# Autodesk Inventor assembly: robot2
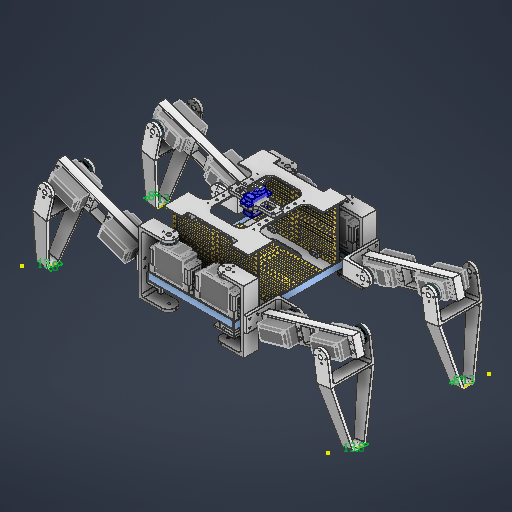
[picture p0: Inventor's stored thumbnail of the model, 512x512]
Saved by Autodesk Inventor 2026.1 (Build 301233000, 233)
## iProperties
Created: 2025-10-04
Part Number: robot2
Document SubType Name: Assembly
Designer: emanuel
Author: emanuel
## Documents named in this file (18)
- C:\Users\emanuel\UnFolder\SpiderRobo\3dmodel\robot2.iam
- C:\Users\emanuel\UnFolder\SpiderRobo\3dmodel\aluminium_profile_1.ipt
- C:\Users\emanuel\UnFolder\SpiderRobo\3dmodel\aluminium_profile_2.ipt
- C:\Users\emanuel\UnFolder\SpiderRobo\3dmodel\mg996r.ipt
- C:\Users\emanuel\UnFolder\SpiderRobo\3dmodel\support_2_servos.ipt
- C:\Users\emanuel\UnFolder\SpiderRobo\3dmodel\servo_disc.ipt
- C:\Users\emanuel\UnFolder\SpiderRobo\3dmodel\servo_support_4.ipt
- C:\Users\emanuel\UnFolder\SpiderRobo\3dmodel\small_bearing.ipt
- C:\Users\emanuel\UnFolder\SpiderRobo\3dmodel\underplate_support_1.ipt
- C:\Users\emanuel\UnFolder\SpiderRobo\3dmodel\bearing_support.ipt
- C:\Users\emanuel\UnFolder\SpiderRobo\3dmodel\C1.ipt
- C:\Users\emanuel\UnFolder\SpiderRobo\3dmodel\femur.ipt
- C:\Users\emanuel\UnFolder\SpiderRobo\3dmodel\L2.ipt
- C:\Users\emanuel\UnFolder\SpiderRobo\3dmodel\smart_calf.ipt
- C:\Users\emanuel\UnFolder\SpiderRobo\3dmodel\yellow_base.iam
- C:\Users\emanuel\UnFolder\SpiderRobo\3dmodel\base.ipt
- C:\Users\emanuel\UnFolder\SpiderRobo\3dmodel\sg90.ipt
- C:\Users\emanuel\UnFolder\SpiderRobo\3dmodel\microservo_support1.ipt
## Components (67 placed, 17 different names)
1. support_2_servos:1 — Mate:9, Flush:5, Mate:10, Mate:25, Flush:13, Flush:14, Mate:26, Flush:15, Flush:16, Mate:27, Flush:17, Flush:18, Mate:28, Flush:19, Flush:20
2. support_2_servos:2 — Mate:7, Flush:4, Mate:8, Mate:20, Mate:21, Flush:6, Mate:22, Flush:7, Flush:8, Mate:23, Flush:9, Flush:10, Mate:24, Flush:11, Flush:12
3. aluminium_profile_1:1 — Mate:3, Mate:4, Flush:2, Mate:5, Flush:3, Mate:7, Mate:43, Flush:22, Mate:46, Flush:25, Mate:128, Mate:134
4. aluminium_profile_1:2 — Mate:1, Mate:2, Flush:1, Mate:6, Mate:9, Mate:44, Flush:23, Mate:45, Flush:27, Mate:127, Mate:132, Mate:137
5. aluminium_profile_2:1 — Mate:5, Mate:6, Flush:3, Flush:4, Mate:8, Flush:26, Flush:28
6. aluminium_profile_2:2 — Mate:1, Mate:2, Flush:1, Mate:3, Mate:4, Flush:2, Flush:5, Mate:10, Flush:21, Flush:24
7. mg996r:1 — Mate:11, Mate:12, Mate:34, Mate:35, Mate:36
8. servo_disc:1 — Mate:11, Mate:12, Mate:49, Mate:51, Mate:52
9. mg996r:2 — Mate:40, Mate:41, Mate:42
10. servo_disc:2 — Mate:79, Mate:80
11. mg996r:3 — Mate:37, Mate:38, Mate:39
12. servo_disc:3 — Mate:69, Mate:70
13. servo_support_4:1 — Mate:28, Flush:19, Flush:20
14. servo_support_4:2 — Mate:26, Flush:15, Flush:16, Mate:34, Mate:35, Mate:36
15. servo_support_4:3 — Mate:27, Flush:17, Flush:18, Mate:31, Mate:32, Mate:33
16. servo_support_4:4 — Mate:25, Flush:13, Flush:14
17. servo_support_4:9 — Mate:20, Mate:21, Flush:6
18. servo_support_4:10 — Mate:23, Flush:9, Flush:10, Mate:37, Mate:38, Mate:39
19. servo_support_4:11 — Mate:22, Flush:7, Flush:8, Mate:40, Mate:41, Mate:42
20. servo_support_4:12 — Mate:24, Flush:11, Flush:12
21. mg996r:4 — Mate:31, Mate:32, Mate:33
22. servo_disc:4 — Mate:77, Mate:78
23. underplate_support_1:1 — Mate:43, Flush:21, Flush:22, Mate:50, Flush:29, Flush:30
24. underplate_support_1:2 — Mate:44, Flush:23, Flush:24
25. underplate_support_1:3 — Mate:46, Flush:25, Flush:26
26. underplate_support_1:4 — Mate:45, Flush:27, Flush:28
27. small_bearing:1 — Mate:49
28. bearing_support:1 — Mate:50, Flush:29, Flush:30
29. C1:1 — Mate:51, Mate:52, Mate:63, Mate:64, Mate:65, Mate:129
30. mg996r:5 — Mate:53, Mate:54, Mate:57, Mate:58, Mate:59
31. femur:1 — Mate:57, Mate:58, Mate:59, Mate:60, Mate:61, Mate:62
32. L2:1 — Mate:63, Mate:64, Mate:65, Mate:119, Mate:120
33. servo_disc:5 — Mate:53, Mate:54, Mate:125, Mate:126
34. mg996r:6 — Mate:60, Mate:61, Mate:62
35. servo_disc:6 — Mate:81, Mate:82
36. L2:4 — Mate:71, Mate:72, Mate:73, Mate:121, Mate:122
37. C1:2 — Mate:69, Mate:70
38. L2:5 — Mate:123, Mate:124
39. C1:3 — Mate:71, Mate:72, Mate:73, Mate:79, Mate:80
40. L2:6 — Mate:125, Mate:126
41. C1:4 — Mate:77, Mate:78
42. smart_calf:1 — Mate:81, Mate:82
43. mg996r:7
44. femur:2
45. servo_disc:7 — Mate:123, Mate:124
46. mg996r:8
47. servo_disc:8
48. smart_calf:2
49. mg996r:9
50. femur:3
51. servo_disc:9 — Mate:121, Mate:122
52. mg996r:10
53. servo_disc:10
54. smart_calf:3
55. mg996r:11
56. femur:4
57. servo_disc:11 — Mate:119, Mate:120
58. mg996r:12
59. servo_disc:12
60. smart_calf:4
61. base:1 — Mate:127, Mate:128, Mate:129, Mate:130, Mate:131, Mate:133, Mate:135, Mate:136, Mate:138
62. yellow_base:1 [sub-assembly] — Mate:130, Mate:131, Mate:132, Mate:139
63. yellow_base:2 [sub-assembly] — Mate:133, Mate:134, Mate:135, Flush:31, Mate:140
64. yellow_base:3 [sub-assembly] — Mate:136, Mate:137, Mate:138
65. base:2 — Mate:139, Flush:31, Mate:140, Mate:144, Mate:145, Mate:146
66. sg90:1 — Mate:141, Mate:142, Mate:143
67. microservo_support1:1 — Mate:141, Mate:142, Mate:143, Mate:144, Mate:145, Mate:146
## Relationships (172: Mate 141, Flush 31)
- Mate:1: aluminium_profile_1:2 ↔ aluminium_profile_2:2
- Mate:2: aluminium_profile_1:2 ↔ aluminium_profile_2:2
- Flush:1: aluminium_profile_1:2 ↔ aluminium_profile_2:2
- Mate:3: aluminium_profile_1:1 ↔ aluminium_profile_2:2
- Mate:4: aluminium_profile_1:1 ↔ aluminium_profile_2:2
- Flush:2: aluminium_profile_1:1 ↔ aluminium_profile_2:2
- Mate:5: aluminium_profile_1:1 ↔ aluminium_profile_2:1
- Mate:6: aluminium_profile_1:2 ↔ aluminium_profile_2:1
- Flush:3: aluminium_profile_1:1 ↔ aluminium_profile_2:1
- Mate:7: support_2_servos:2 ↔ aluminium_profile_1:1
- Flush:4: support_2_servos:2 ↔ aluminium_profile_2:1
- Mate:8: support_2_servos:2 ↔ aluminium_profile_2:1
- Mate:9: support_2_servos:1 ↔ aluminium_profile_1:2
- Flush:5: support_2_servos:1 ↔ aluminium_profile_2:2
- Mate:10: support_2_servos:1 ↔ aluminium_profile_2:2
- Mate:11: mg996r:1 ↔ servo_disc:1
- Mate:12: mg996r:1 ↔ servo_disc:1
- [Mate]: mg996r:2 ↔ servo_disc:2
- [Mate]: mg996r:2 ↔ servo_disc:2
- [Mate]: mg996r:3 ↔ servo_disc:3
- [Mate]: mg996r:3 ↔ servo_disc:3
- Mate:20: support_2_servos:2 ↔ servo_support_4:9
- Mate:21: support_2_servos:2 ↔ servo_support_4:9
- Flush:6: support_2_servos:2 ↔ servo_support_4:9
- Mate:22: support_2_servos:2 ↔ servo_support_4:11
- Flush:7: support_2_servos:2 ↔ servo_support_4:11
- Flush:8: support_2_servos:2 ↔ servo_support_4:11
- Mate:23: support_2_servos:2 ↔ servo_support_4:10
- Flush:9: support_2_servos:2 ↔ servo_support_4:10
- Flush:10: support_2_servos:2 ↔ servo_support_4:10
- Mate:24: support_2_servos:2 ↔ servo_support_4:12
- Flush:11: support_2_servos:2 ↔ servo_support_4:12
- Flush:12: support_2_servos:2 ↔ servo_support_4:12
- Mate:25: support_2_servos:1 ↔ servo_support_4:4
- Flush:13: support_2_servos:1 ↔ servo_support_4:4
- Flush:14: support_2_servos:1 ↔ servo_support_4:4
- Mate:26: support_2_servos:1 ↔ servo_support_4:2
- Flush:15: support_2_servos:1 ↔ servo_support_4:2
- Flush:16: support_2_servos:1 ↔ servo_support_4:2
- Mate:27: support_2_servos:1 ↔ servo_support_4:3
- Flush:17: support_2_servos:1 ↔ servo_support_4:3
- Flush:18: support_2_servos:1 ↔ servo_support_4:3
- Mate:28: support_2_servos:1 ↔ servo_support_4:1
- Flush:19: support_2_servos:1 ↔ servo_support_4:1
- Flush:20: support_2_servos:1 ↔ servo_support_4:1
- [Mate]: mg996r:4 ↔ servo_disc:4
- [Mate]: mg996r:4 ↔ servo_disc:4
- Mate:31: servo_support_4:3 ↔ mg996r:4
- Mate:32: servo_support_4:3 ↔ mg996r:4
- Mate:33: servo_support_4:3 ↔ mg996r:4
- Mate:34: mg996r:1 ↔ servo_support_4:2
- Mate:35: mg996r:1 ↔ servo_support_4:2
- Mate:36: mg996r:1 ↔ servo_support_4:2
- Mate:37: mg996r:3 ↔ servo_support_4:10
- Mate:38: mg996r:3 ↔ servo_support_4:10
- Mate:39: mg996r:3 ↔ servo_support_4:10
- Mate:40: mg996r:2 ↔ servo_support_4:11
- Mate:41: mg996r:2 ↔ servo_support_4:11
- Mate:42: mg996r:2 ↔ servo_support_4:11
- Mate:43: aluminium_profile_1:1 ↔ underplate_support_1:1
- Flush:21: aluminium_profile_2:2 ↔ underplate_support_1:1
- Flush:22: aluminium_profile_1:1 ↔ underplate_support_1:1
- Mate:44: aluminium_profile_1:2 ↔ underplate_support_1:2
- Flush:23: aluminium_profile_1:2 ↔ underplate_support_1:2
- Flush:24: aluminium_profile_2:2 ↔ underplate_support_1:2
- Mate:45: aluminium_profile_1:2 ↔ underplate_support_1:4
- Mate:46: aluminium_profile_1:1 ↔ underplate_support_1:3
- Flush:25: aluminium_profile_1:1 ↔ underplate_support_1:3
- Flush:26: aluminium_profile_2:1 ↔ underplate_support_1:3
- Flush:27: aluminium_profile_1:2 ↔ underplate_support_1:4
- Flush:28: aluminium_profile_2:1 ↔ underplate_support_1:4
- Mate:49: servo_disc:1 ↔ small_bearing:1
- Mate:50: underplate_support_1:1 ↔ bearing_support:1
- Flush:29: underplate_support_1:1 ↔ bearing_support:1
- Flush:30: underplate_support_1:1 ↔ bearing_support:1
- Mate:51: servo_disc:1 ↔ C1:1
- Mate:52: servo_disc:1 ↔ C1:1
- Mate:53: mg996r:5 ↔ servo_disc:5
- Mate:54: mg996r:5 ↔ servo_disc:5
- [Mate]: mg996r:6 ↔ servo_disc:6
- [Mate]: mg996r:6 ↔ servo_disc:6
- Mate:57: mg996r:5 ↔ femur:1
- Mate:58: mg996r:5 ↔ femur:1
- Mate:59: mg996r:5 ↔ femur:1
- Mate:60: femur:1 ↔ mg996r:6
- Mate:61: femur:1 ↔ mg996r:6
- Mate:62: femur:1 ↔ mg996r:6
- Mate:63: C1:1 ↔ L2:1
- Mate:64: C1:1 ↔ L2:1
- Mate:65: C1:1 ↔ L2:1
- [Mate]: C1:2 ↔ L2:5
- [Mate]: C1:2 ↔ L2:5
- [Mate]: C1:2 ↔ L2:5
- Mate:69: servo_disc:3 ↔ C1:2
- Mate:70: servo_disc:3 ↔ C1:2
- Mate:71: L2:4 ↔ C1:3
- Mate:72: L2:4 ↔ C1:3
- Mate:73: L2:4 ↔ C1:3
- [Mate]: L2:6 ↔ C1:4
- [Mate]: L2:6 ↔ C1:4
- [Mate]: L2:6 ↔ C1:4
- Mate:77: servo_disc:4 ↔ C1:4
- Mate:78: servo_disc:4 ↔ C1:4
- Mate:79: servo_disc:2 ↔ C1:3
- Mate:80: servo_disc:2 ↔ C1:3
- Mate:81: servo_disc:6 ↔ smart_calf:1
- Mate:82: servo_disc:6 ↔ smart_calf:1
- [Mate]: mg996r:7 ↔ servo_disc:7
- [Mate]: mg996r:7 ↔ servo_disc:7
- [Mate]: mg996r:8 ↔ servo_disc:8
- [Mate]: mg996r:8 ↔ servo_disc:8
- [Mate]: mg996r:7 ↔ femur:2
- [Mate]: mg996r:7 ↔ femur:2
- [Mate]: mg996r:7 ↔ femur:2
- [Mate]: femur:2 ↔ mg996r:8
- [Mate]: femur:2 ↔ mg996r:8
- [Mate]: femur:2 ↔ mg996r:8
- [Mate]: servo_disc:8 ↔ smart_calf:2
- [Mate]: servo_disc:8 ↔ smart_calf:2
- [Mate]: mg996r:9 ↔ servo_disc:9
- [Mate]: mg996r:9 ↔ servo_disc:9
- [Mate]: mg996r:10 ↔ servo_disc:10
- [Mate]: mg996r:10 ↔ servo_disc:10
- [Mate]: mg996r:9 ↔ femur:3
- [Mate]: mg996r:9 ↔ femur:3
- [Mate]: mg996r:9 ↔ femur:3
- [Mate]: femur:3 ↔ mg996r:10
- [Mate]: femur:3 ↔ mg996r:10
- [Mate]: femur:3 ↔ mg996r:10
- [Mate]: servo_disc:10 ↔ smart_calf:3
- [Mate]: servo_disc:10 ↔ smart_calf:3
- [Mate]: mg996r:11 ↔ servo_disc:11
- [Mate]: mg996r:11 ↔ servo_disc:11
- [Mate]: mg996r:12 ↔ servo_disc:12
- [Mate]: mg996r:12 ↔ servo_disc:12
- [Mate]: mg996r:11 ↔ femur:4
- [Mate]: mg996r:11 ↔ femur:4
- [Mate]: mg996r:11 ↔ femur:4
- [Mate]: femur:4 ↔ mg996r:12
- [Mate]: femur:4 ↔ mg996r:12
- [Mate]: femur:4 ↔ mg996r:12
- [Mate]: servo_disc:12 ↔ smart_calf:4
- [Mate]: servo_disc:12 ↔ smart_calf:4
- Mate:119: L2:1 ↔ servo_disc:11
- Mate:120: L2:1 ↔ servo_disc:11
- Mate:121: L2:4 ↔ servo_disc:9
- Mate:122: L2:4 ↔ servo_disc:9
- Mate:123: L2:5 ↔ servo_disc:7
- Mate:124: L2:5 ↔ servo_disc:7
- Mate:125: servo_disc:5 ↔ L2:6
- Mate:126: servo_disc:5 ↔ L2:6
- Mate:127: aluminium_profile_1:2 ↔ base:1
- Mate:128: aluminium_profile_1:1 ↔ base:1
- Mate:129: C1:1 ↔ base:1
- Mate:130: base:1 ↔ yellow_base:1
- Mate:131: base:1 ↔ yellow_base:1
- Mate:132: aluminium_profile_1:2 ↔ yellow_base:1
- Mate:133: base:1 ↔ yellow_base:2
- Mate:134: aluminium_profile_1:1 ↔ yellow_base:2
- Mate:135: base:1 ↔ yellow_base:2
- Mate:136: base:1 ↔ yellow_base:3
- Mate:137: aluminium_profile_1:2 ↔ yellow_base:3
- Mate:138: base:1 ↔ yellow_base:3
- Mate:139: yellow_base:1 ↔ base:2
- Flush:31: yellow_base:2 ↔ base:2
- Mate:140: yellow_base:2 ↔ base:2
- Mate:141: sg90:1 ↔ microservo_support1:1
- Mate:142: sg90:1 ↔ microservo_support1:1
- Mate:143: sg90:1 ↔ microservo_support1:1
- Mate:144: base:2 ↔ microservo_support1:1
- Mate:145: base:2 ↔ microservo_support1:1
- Mate:146: base:2 ↔ microservo_support1:1
## Named parameters: d49_d47 = 0 mm, d50_d48 = 0 mm, d51_d47 = 0 mm, d52_d48 = 0 mm, d80_d47 = 0 mm, d81_d48 = 0 mm, d127_d125 = 0 mm, d128_d126 = 0 mm, d138_d135 = 0 mm, d139_d136 = 0 mm, d140_d137 = 0 mm, d146_d143 = 0 mm, d147_d144 = 0 mm, d148_d145 = 0 mm, d155_d153 = 0 mm, d156_d125 = 0 mm, d157_d126 = 0 mm, d158_d127_d125 = 0 mm, d159_d128_d126 = 0 mm, d160_d129 = 0 mm, d161_d130 = 0 mm, d162_d131 = 0 mm, d163_d132 = 0 mm, d164_d133 = 0 mm, d165_d134 = 0 mm, d166_d154 = 0 mm, d167_d153 = 0 mm, d168_d125 = 0 mm, d169_d126 = 0 mm, d170_d127_d125 = 0 mm, d171_d128_d126 = 0 mm, d172_d129 = 0 mm, d173_d130 = 0 mm, d174_d131 = 0 mm, d175_d132 = 0 mm, d176_d133 = 0 mm, d177_d134 = 0 mm, d178_d154 = 0 mm, d179_d153 = 0 mm, d180_d125 = 0 mm, d181_d126 = 0 mm, d182_d127_d125 = 0 mm, d183_d128_d126 = 0 mm, d184_d129 = 0 mm, d185_d130 = 0 mm, d186_d131 = 0 mm, d187_d132 = 0 mm, d188_d133 = 0 mm, d189_d134 = 0 mm, d190_d154 = 0 mm
